# Autodesk Inventor assembly: HS 48T Gear, No Insert, Lathe
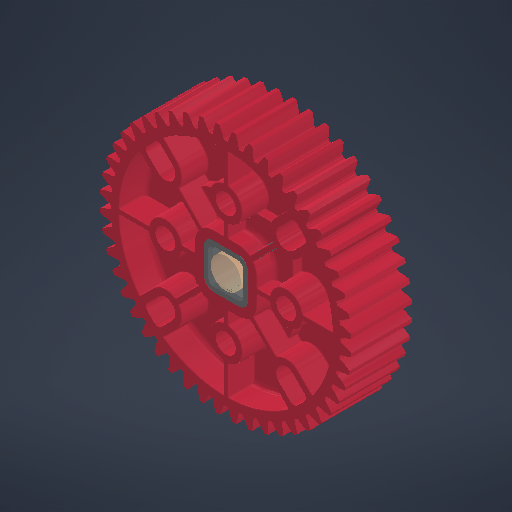
[picture p0: Inventor's stored thumbnail of the model, 512x512]
Saved by Autodesk Inventor 2026.1 (Build 301233000, 233)
## iProperties
Created: 2022-08-02
Document SubType Name: Assembly
Designer: ylu12
Author: ylu12
## Documents named in this file (3)
- C:\3284b-cad-2025\Library\Custom Parts\HS 48T Gear, No Insert, Lathe.iam
- C:\3284b-cad-2025\Library\VEX-CAD-Inventor-1.4.2\Motion\Gears\Reference Files\HS 48T Gear, No Insert.ipt
- C:\3284b-cad-2025\Library\VEX-CAD-Inventor-1.4.2\Motion\Gears\HS Gear.iam
## Components (1 placed, 1 different names)
1. 48T — Flush:6, Mate:11, Mate:12
## Relationships (3: Mate 2, Flush 1)
- Flush:6: 48T
- Mate:11: 48T
- Mate:12: 48T
